# Autodesk Inventor assembly: thermal
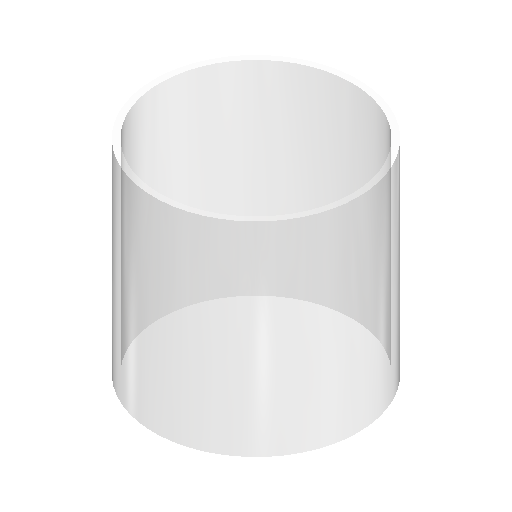
[picture p0: Inventor's stored thumbnail of the model, 512x512]
Saved by Autodesk Inventor 2026.2 (Build 302298010, 298A)
## iProperties
Created: 2026-04-29
Part Number: thermal
Document SubType Name: Assembly
Designer: danie
Author: danie
## Documents named in this file (2)
- C:\Users\danie\OneDrive\Documentos\Inventor\Arbol\V4\V4\thermal.iam
- C:\Users\danie\OneDrive\Documentos\Inventor\Arbol\V4\V4\Chasis\Tuberia.ipt
## Components (1 placed, 1 different names)
1. Tuberia:1 — Mate:1, Flush:1, Mate:2
## Relationships (3: Mate 2, Flush 1)
- Mate:1: Tuberia:1
- Flush:1: Tuberia:1
- Mate:2: Tuberia:1
